# Autodesk Inventor assembly: Complete Reflow Oven
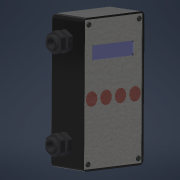
[picture p0: Inventor's stored thumbnail of the model, 180x180]
Saved by Autodesk Inventor 2021 (Build 250183000, 183)
## iProperties
Created: 2014-08-04
Part Number: Complete Reflow Oven
Document SubType Name: Assembly
Designer: simon
Author: simon
## Documents named in this file (9)
- D:\Develop\Reflow_Oven_USB\Inventor\Complete Reflow Oven.iam
- D:\Develop\Reflow_Oven_USB\Inventor\1591D Box.ipt
- D:\Develop\Reflow_Oven_USB\Inventor\Imported Components\gn 16 cable gland\gn 16 cable gland.ipt
- D:\Develop\Reflow_Oven_USB\Inventor\Polycarbonate Facia.ipt
- D:\Develop\Reflow_Oven_USB\Inventor\Imported Components\NHD-0216HZ\NHD-0216HZ.ipt
- D:\Develop\Reflow_Oven_USB\Inventor\Imported Components\Reflow Front\Reflow Front.iam
- D:\Develop\Reflow_Oven_USB\Inventor\Imported Components\Reflow MCU\Reflow MCU.iam
- C:\Users\simon\Documents\Inventor\Content Center Files\R2021\en-US\ISO 7380-1\ISO 7380-1 - M3 x 8.ipt
- D:\Develop\Reflow_Oven_USB\Inventor\Paper Sheet.ipt
## Components (12 placed, 8 different names)
1. 1591D Box:1 — Mate:2, Mate:4, Angle:1, Angle:2, Insert:1, Insert:2, Insert:11, Insert:12
2. gn 16 cable gland:1 — Mate:2, Angle:1, Insert:11
3. gn 16 cable gland:2 — Mate:4, Angle:2, Insert:12
4. Polycarbonate Facia:1 — Insert:5, Insert:6, Insert:7, Insert:8, Insert:9, Insert:10
5. NHD-0216HZ:1 — Mate:8, Mate:10, Mate:14
6. Reflow Front:1 [sub-assembly] — Insert:1, Insert:2, Mate:8, Mate:10, Mate:11, Mate:12, Mate:13, Insert:3, Insert:4
7. Reflow MCU:1 [sub-assembly] — Mate:11, Mate:12, Mate:13
8. Paper Sheet:1 — Insert:3, Insert:4, Insert:5, Insert:6, Mate:14
9. ISO 7380-1 M3 x 8:1 — Insert:7
10. ISO 7380-1 M3 x 8:2 — Insert:8
11. ISO 7380-1 M3 x 8:3 — Insert:9
12. ISO 7380-1 M3 x 8:4 — Insert:10
## Relationships (22: Insert 12, Mate 8, Angle 2)
- Mate:2: 1591D Box:1 ↔ gn 16 cable gland:1
- Mate:4: 1591D Box:1 ↔ gn 16 cable gland:2
- Angle:1 (90 deg): 1591D Box:1 ↔ gn 16 cable gland:1
- Angle:2 (90 deg): 1591D Box:1 ↔ gn 16 cable gland:2
- Insert:1: 1591D Box:1 ↔ Reflow Front:1
- Insert:2: 1591D Box:1 ↔ Reflow Front:1
- Mate:8: NHD-0216HZ:1 ↔ Reflow Front:1
- Mate:10: NHD-0216HZ:1 ↔ Reflow Front:1
- Mate:11: Reflow Front:1 ↔ Reflow MCU:1
- Mate:12: Reflow Front:1 ↔ Reflow MCU:1
- Mate:13: Reflow Front:1 ↔ Reflow MCU:1
- Insert:3: Reflow Front:1 ↔ Paper Sheet:1
- Insert:4: Reflow Front:1 ↔ Paper Sheet:1
- Insert:5: Polycarbonate Facia:1 ↔ Paper Sheet:1
- Insert:6: Polycarbonate Facia:1 ↔ Paper Sheet:1
- Insert:7: Polycarbonate Facia:1 ↔ ISO 7380-1 M3 x 8:1
- Insert:8: Polycarbonate Facia:1 ↔ ISO 7380-1 M3 x 8:2
- Insert:9: Polycarbonate Facia:1 ↔ ISO 7380-1 M3 x 8:3
- Insert:10: Polycarbonate Facia:1 ↔ ISO 7380-1 M3 x 8:4
- Mate:14: NHD-0216HZ:1 ↔ Paper Sheet:1
- Insert:11: 1591D Box:1 ↔ gn 16 cable gland:1
- Insert:12: 1591D Box:1 ↔ gn 16 cable gland:2
